# Autodesk Inventor assembly: UpperArm
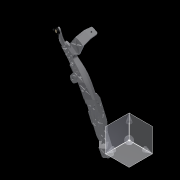
[picture p0: Inventor's stored thumbnail of the model, 180x180]
Saved by Autodesk Inventor 2015 SP1 (Build 190203100, 203)
## iProperties
Created: 2014-08-07
Part Number: UpperArm
Document SubType Name: Assembly
Designer: Val
Mass: 392.322 g
Surface Area: 590.202 cm^2
Volume: 151.879 cm^3
Density: 2.58312 g/cm^3
Author: Val
## Documents named in this file (7)
- E:\Exo\Models\3D\UpperArmRight.iam
- E:\Exo\Models\3D\UpperArmRight.ipt
- E:\Exo\Models\3D\UpperArmShoulderRight.ipt
- E:\Exo\Models\3D\UpperArmTricepRight.ipt
- E:\Exo\Models\3D\UpperArmConnectorRight.ipt
- E:\Exo\Models\3D\External\BearingBall.ipt
- E:\Exo\Models\3D\External\BearingBody.ipt
## Components (6 placed, 6 different names)
1. UpperArmRight:1 — Mate:1, Mate:2, Mate:3, Mate:5, Mate:6, Mate:7, Mate:13
2. UpperArmShoulderRight:1 — Mate:1, Mate:2, Mate:3
3. UpperArmTricepRight:1 — Mate:5, Mate:6, Mate:7
4. UpperArmTwistConnectorRight:1 — Mate:13, Mate:14
5. BearingBall:1 — Mate:12, Mate:14
6. BearingBody:1 — Mate:12
## Relationships (9: Mate 9)
- Mate:1: UpperArmRight:1 ↔ UpperArmShoulderRight:1
- Mate:2: UpperArmRight:1 ↔ UpperArmShoulderRight:1
- Mate:3: UpperArmRight:1 ↔ UpperArmShoulderRight:1
- Mate:5: UpperArmRight:1 ↔ UpperArmTricepRight:1
- Mate:6: UpperArmRight:1 ↔ UpperArmTricepRight:1
- Mate:7: UpperArmRight:1 ↔ UpperArmTricepRight:1
- Mate:12: BearingBall:1 ↔ BearingBody:1
- Mate:13: UpperArmRight:1 ↔ UpperArmTwistConnectorRight:1
- Mate:14: UpperArmTwistConnectorRight:1 ↔ BearingBall:1
